# Autodesk Inventor assembly: Assembly3
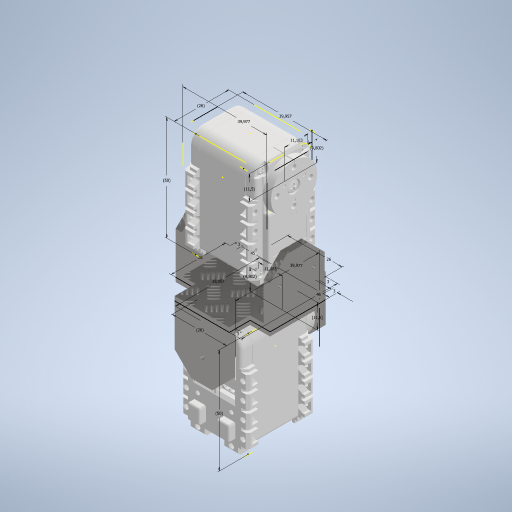
[picture p0: Inventor's stored thumbnail of the model, 512x512]
Saved by Autodesk Inventor 2024 (Build 280153000, 153)
## iProperties
Created: 2024-02-16
Part Number: Assembly3
Document SubType Name: Assembly
Designer: kamil
Author: kamil
## Documents named in this file (3)
- D:\Projects\Robotics\Hexapod\Assembly3.iam
- D:\Projects\Robotics\Hexapod\first_junction.ipt
- D:\Projects\Robotics\Hexapod\AX-12A\AX-12A.iam
## Components (3 placed, 2 different names)
1. first_junction:1 — Mate:1, Mate:2, Mate:3, Mate:4, Mate:5, Mate:6, Mate:7
2. AX-12A:1 [sub-assembly] — Mate:1, Mate:2, Mate:3, Mate:4
3. AX-12A:2 [sub-assembly] — Mate:5, Mate:6, Mate:7
## Relationships (7: Mate 7)
- Mate:1: first_junction:1 ↔ AX-12A:1
- Mate:2: first_junction:1 ↔ AX-12A:1
- Mate:3: first_junction:1 ↔ AX-12A:1
- Mate:4: first_junction:1 ↔ AX-12A:1
- Mate:5: first_junction:1 ↔ AX-12A:2
- Mate:6: first_junction:1 ↔ AX-12A:2
- Mate:7: first_junction:1 ↔ AX-12A:2
